# Autodesk Inventor assembly: Elevador
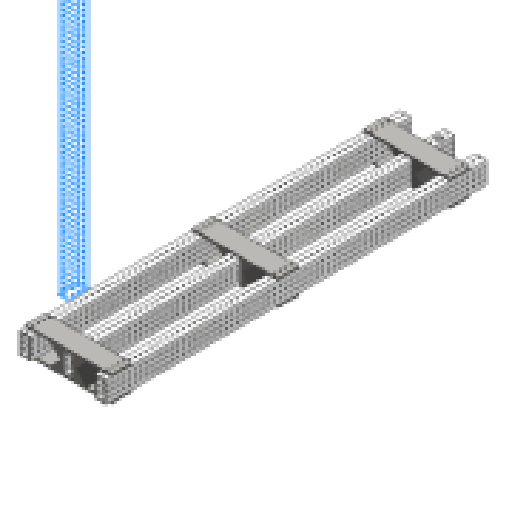
[picture p0: Inventor's stored thumbnail of the model, 512x512]
Saved by Autodesk Inventor 2027.1 (Build 311270010, 270A)
## iProperties
Created: 2026-05-13
Part Number: Elevador
Document SubType Name: Assembly
Designer: djair.oliveira
Author: djair.oliveira
## Documents named in this file (4)
- C:\Users\djair.oliveira\Documents\GitHub\MT_2026\CAD\Model C\Elevador\Elevador.iam
- C:\Users\djair.oliveira\Documents\GitHub\MT_2026\CAD\Model C\Elevador\Chapa Guia - Elevador.ipt
- C:\Users\djair.oliveira\Documents\GitHub\MT_2026\CAD\Model C\Elevador\Forja - Base1 Elevador.ipt
- C:\Users\djair.oliveira\Documents\GitHub\MT_2026\CAD\Model C\Elevador\Forja - Move Elevador.ipt
## Components (9 placed, 3 different names)
1. Chapa Guia - Elevador:1 — Coincidente:1, Coincidente:2, Coincidente:3, Coincidente:4
2. Chapa Guia - Elevador:2 — Coincidente:5, Coincidente:6, Coincidente:7, Alinhado:3
3. Chapa Guia - Elevador:3 — Coincidente:8, Coincidente:9, Coincidente:10, Coincidente:21
4. Chapa Guia - Elevador:4 — Coincidente:11, Coincidente:12, Coincidente:13
5. Forja - Base1 Elevador:1 — Alinhado:1, Alinhado:2, Coincidente:1, Coincidente:2, Coincidente:3, Coincidente:7, Coincidente:10, Coincidente:13, Coincidente:14, Coincidente:15, Coincidente:17, Coincidente:18
6. Forja - Base1 Elevador:2 — Alinhado:1, Alinhado:2, Coincidente:4, Coincidente:5, Coincidente:6, Coincidente:8, Coincidente:9, Coincidente:11, Coincidente:12, Coincidente:16, Coincidente:19
7. Chapa Guia - Elevador:5 — Coincidente:17, Coincidente:18, Coincidente:19, Coincidente:20
8. Chapa Guia - Elevador:6 — Coincidente:14, Coincidente:15, Coincidente:16
9. Forja - Move Elevador:1 — Coincidente:20, Coincidente:21, Alinhado:3
## Relationships (24: Mate 21, Flush 3)
- Alinhado:1 [Flush]: Forja - Base1 Elevador:1 ↔ Forja - Base1 Elevador:2
- Alinhado:2 [Flush]: Forja - Base1 Elevador:1 ↔ Forja - Base1 Elevador:2
- Coincidente:1 [Mate]: Chapa Guia - Elevador:1 ↔ Forja - Base1 Elevador:1
- Coincidente:2 [Mate]: Chapa Guia - Elevador:1 ↔ Forja - Base1 Elevador:1
- Coincidente:3 [Mate]: Chapa Guia - Elevador:1 ↔ Forja - Base1 Elevador:1
- Coincidente:4 [Mate]: Chapa Guia - Elevador:1 ↔ Forja - Base1 Elevador:2
- Coincidente:5 [Mate]: Chapa Guia - Elevador:2 ↔ Forja - Base1 Elevador:2
- Coincidente:6 [Mate]: Chapa Guia - Elevador:2 ↔ Forja - Base1 Elevador:2
- Coincidente:7 [Mate]: Chapa Guia - Elevador:2 ↔ Forja - Base1 Elevador:1
- Coincidente:8 [Mate]: Chapa Guia - Elevador:3 ↔ Forja - Base1 Elevador:2
- Coincidente:9 [Mate]: Chapa Guia - Elevador:3 ↔ Forja - Base1 Elevador:2
- Coincidente:10 [Mate]: Chapa Guia - Elevador:3 ↔ Forja - Base1 Elevador:1
- Coincidente:11 [Mate]: Chapa Guia - Elevador:4 ↔ Forja - Base1 Elevador:2
- Coincidente:12 [Mate]: Chapa Guia - Elevador:4 ↔ Forja - Base1 Elevador:2
- Coincidente:13 [Mate]: Chapa Guia - Elevador:4 ↔ Forja - Base1 Elevador:1
- Coincidente:14 [Mate]: Forja - Base1 Elevador:1 ↔ Chapa Guia - Elevador:6
- Coincidente:15 [Mate]: Forja - Base1 Elevador:1 ↔ Chapa Guia - Elevador:6
- Coincidente:16 [Mate]: Forja - Base1 Elevador:2 ↔ Chapa Guia - Elevador:6
- Coincidente:17 [Mate]: Forja - Base1 Elevador:1 ↔ Chapa Guia - Elevador:5
- Coincidente:18 [Mate]: Forja - Base1 Elevador:1 ↔ Chapa Guia - Elevador:5
- Coincidente:19 [Mate]: Forja - Base1 Elevador:2 ↔ Chapa Guia - Elevador:5
- Coincidente:20 [Mate]: Chapa Guia - Elevador:5 ↔ Forja - Move Elevador:1
- Coincidente:21 [Mate]: Chapa Guia - Elevador:3 ↔ Forja - Move Elevador:1
- Alinhado:3 [Flush]: Chapa Guia - Elevador:2 ↔ Forja - Move Elevador:1
